# Autodesk Inventor assembly: PneummaticActuator
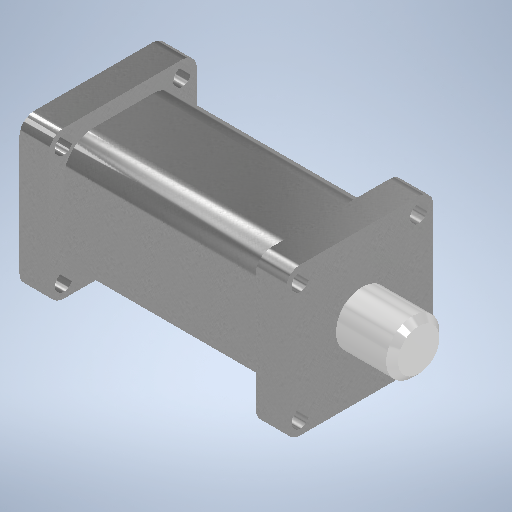
[picture p0: Inventor's stored thumbnail of the model, 512x512]
Saved by Autodesk Inventor 2025.1 (Build 291241000, 241)
## iProperties
Created: 2025-02-26
Part Number: PneummaticActuator
Document SubType Name: Assembly
Designer: yovan
Author: yovan
## Documents named in this file (3)
- C:\Users\yovan\Desktop\APM\ausol-apm.github.io\project\Design and simulation\Inventor\NXModeling\PneumaticActuator\PneummaticActuator.iam
- C:\Users\yovan\Desktop\APM\ausol-apm.github.io\project\Design and simulation\Inventor\NXModeling\PneumaticActuator\Contenedor.ipt
- C:\Users\yovan\Desktop\APM\ausol-apm.github.io\project\Design and simulation\Inventor\NXModeling\PneumaticActuator\Embolo.ipt
## Components (2 placed, 2 different names)
1. Contenedor:1 — Mate:2
2. Embolo:1 — Mate:2
## Relationships (1: Mate 1)
- Mate:2: Contenedor:1 ↔ Embolo:1
